# Autodesk Inventor assembly: Jack lift
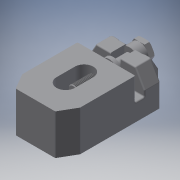
[picture p0: Inventor's stored thumbnail of the model, 180x180]
Saved by Autodesk Inventor 2017.2 (Build 212233000, 233)
## iProperties
Created: 2017-03-23
Part Number: Jack lift
Document SubType Name: Assembly
Designer: 196918
Author: 196918
## Documents named in this file (4)
- C:\Users\196918\Desktop\Jack lift.iam
- C:\Users\196918\Desktop\Base.ipt
- C:\Users\196918\Desktop\Wedge.ipt
- C:\Users\196918\Desktop\Wedge_Screw.ipt
## Components (3 placed, 3 different names)
1. Base:1 — Rigid:2
2. Wedge:1 — Rigid:1, Rigid:2
3. Wedge_Screw:1 — Rigid:1
## Relationships (2: WeldJoint 2)
- Rigid:1 [WeldJoint]: Wedge:1 ↔ Wedge_Screw:1
- Rigid:2 [WeldJoint]: Base:1 ↔ Wedge:1
